# Autodesk Inventor assembly: ASY TRM 050 shaft
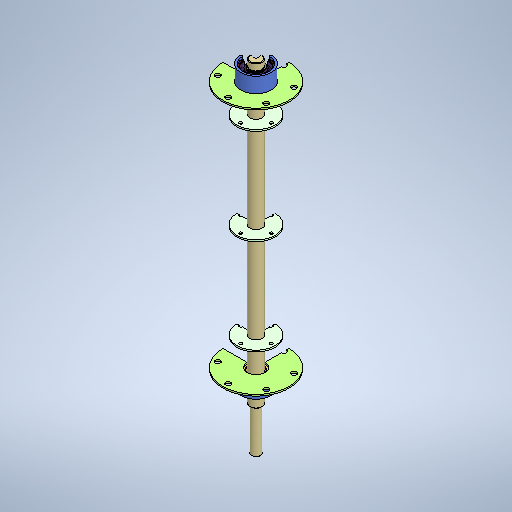
[picture p0: Inventor's stored thumbnail of the model, 512x512]
Saved by Autodesk Inventor 2025 (Build 290162010, 162A)
## iProperties
Created: 2024-09-11
Part Number: ASY TRM 050 shaft
Document SubType Name: Assembly
Designer: pokla
Author: pokla
## Documents named in this file (5)
- C:\Users\pokla\Documents\Inventor\BSH_Beshkino_bio_tank\ASY TRM 050 shaft.iam
- C:\Users\pokla\Documents\Inventor\BSH_Beshkino_bio_tank\TRM 028 main shaft.ipt
- C:\Users\pokla\Documents\Inventor\BSH_Beshkino_bio_tank\TRM 029 coupling ring.ipt
- C:\Users\pokla\Documents\Inventor\BSH_Beshkino_bio_tank\Content Center Files\en-US\CNS 9074(1)\CNS 9074 - 24 x 1,2(2).ipt
- C:\Users\pokla\Documents\Inventor\BSH_Beshkino_bio_tank\ASY TRM 040 seal.iam
## Components (8 placed, 4 different names)
1. ASY TRM 040 seal:1 [sub-assembly] — Rotational:1
2. ASY TRM 040 seal:2 [sub-assembly] — Rotational:2
3. TRM 028 main shaft:1 — Rigid:2, Mate:1, Mate:2, Mate:3, Mate:4, Rotational:1, Rotational:2
4. TRM 029 coupling ring:1
5. TRM 029 coupling ring:2 — Rigid:2
6. TRM 029 coupling ring:3
7. CNS 9074 24 x 1,2:1 — Mate:1, Mate:2
8. CNS 9074 24 x 1,2:2 — Mate:3, Mate:4
## Relationships (10: Mate 4, WeldJoint 3, RevoluteJoint 2, Flush 1)
- [WeldJoint] (-283.5 mm): TRM 028 main shaft:1 ↔ TRM 029 coupling ring:3
- Rigid:2 [WeldJoint] (-95 mm): TRM 028 main shaft:1 ↔ TRM 029 coupling ring:2
- [WeldJoint] (-472 mm): TRM 028 main shaft:1 ↔ TRM 029 coupling ring:1
- Mate:1: TRM 028 main shaft:1 ↔ CNS 9074 24 x 1,2:1
- Mate:2: TRM 028 main shaft:1 ↔ CNS 9074 24 x 1,2:1
- Mate:3: TRM 028 main shaft:1 ↔ CNS 9074 24 x 1,2:2
- Mate:4: TRM 028 main shaft:1 ↔ CNS 9074 24 x 1,2:2
- [Flush] (1 mm): ASY TRM 040 seal:2 ↔ TRM 028 main shaft:1
- Rotational:1 [RevoluteJoint] (-121 mm): ASY TRM 040 seal:1 ↔ TRM 028 main shaft:1
- Rotational:2 [RevoluteJoint] (-16 mm): ASY TRM 040 seal:2 ↔ TRM 028 main shaft:1
